# Autodesk Inventor assembly: sestava tělo estonsko s plechem
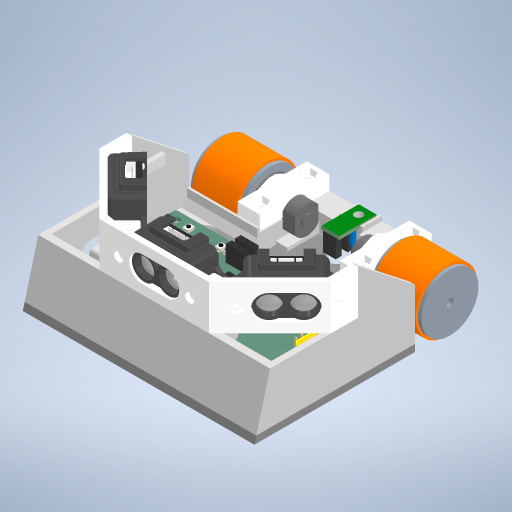
[picture p0: Inventor's stored thumbnail of the model, 512x512]
Saved by Autodesk Inventor 2024 (Build 280153000, 153)
## iProperties
Created: 2023-11-06
Part Number: sestava tělo estonsko s plechem
Document SubType Name: Assembly
Designer: jaryj
Author: jaryj
## Documents named in this file (9)
- C:\Users\Simak\OneDrive\Dokumenty\GitHub\RoboCop\- 3D -\wip\Tělo s plechem\sestava tělo estonsko s plechem.iam
- C:\Users\Simak\OneDrive\Dokumenty\GitHub\RoboCop\- 3D -\wip\Tělo s plechem\tělo estonsko s plechem.ipt
- C:\Users\Simak\OneDrive\Dokumenty\GitHub\RoboCop\- 3D -\el._parts\GA12-N20_Motor.ipt
- C:\Users\Simak\OneDrive\Dokumenty\GitHub\RoboCop\- 3D -\mech._parts\wheel+silicon.ipt
- C:\Users\Simak\OneDrive\Dokumenty\GitHub\RoboCop\- 3D -\wip\Sestava TF-Luna a držáku.iam
- C:\Users\Simak\OneDrive\Dokumenty\GitHub\RoboCop\- 3D -\mech._parts\plech.ipt
- C:\Users\Simak\OneDrive\Dokumenty\GitHub\RoboCop\- 3D -\el._parts\sumec_smd.iam
- C:\Users\Simak\OneDrive\Dokumenty\GitHub\RoboCop\- 3D -\mech._parts\motor_C_clamp_nutt.ipt
- C:\Users\Simak\OneDrive\Dokumenty\GitHub\RoboCop\- 3D -\el._parts\qre_module.ipt
## Components (11 placed, 8 different names)
1. tělo estonsko s plechem:1 — Vložit:2, Proti sobě:1, Vložit:3, Proti sobě:2, Proti sobě:5, Proti sobě:6, Proti sobě:10, Stejný směr:1, Proti sobě:11, Stejný směr:2, Proti sobě:12, Stejný směr:3, Proti sobě:13, Vložit:4, Vložit:5, Vložit:6, Vložit:7, Proti sobě:17, Vložit:8
2. GA12-N20_Motor:1 — Vložit:2, Proti sobě:1, Proti sobě:3, Proti sobě:14
3. GA12-N20_Motor:2 — Vložit:3, Proti sobě:2, Proti sobě:4, Proti sobě:15
4. wheel+silicon:1 — Proti sobě:4, Proti sobě:5
5. wheel+silicon:2 — Proti sobě:3, Proti sobě:6
6. Sestava TF-Luna a držáku:1 [sub-assembly] — Proti sobě:10, Stejný směr:1, Proti sobě:11
7. plech:1 — Stejný směr:2, Proti sobě:12, Stejný směr:3
8. sumec_smd:1 [sub-assembly] — Proti sobě:13, Vložit:4, Vložit:5
9. motor_C_clamp_nutt:1 — Proti sobě:15, Vložit:7
10. motor_C_clamp_nutt:2 — Proti sobě:14, Vložit:6
11. qre_module:1 — Proti sobě:17, Vložit:8
## Relationships (23: Mate 13, Insert 7, Flush 3)
- Vložit:2 [Insert]: tělo estonsko s plechem:1 ↔ GA12-N20_Motor:1
- Proti sobě:1 [Mate]: tělo estonsko s plechem:1 ↔ GA12-N20_Motor:1
- Vložit:3 [Insert]: tělo estonsko s plechem:1 ↔ GA12-N20_Motor:2
- Proti sobě:2 [Mate]: tělo estonsko s plechem:1 ↔ GA12-N20_Motor:2
- Proti sobě:3 [Mate]: GA12-N20_Motor:1 ↔ wheel+silicon:2
- Proti sobě:4 [Mate]: GA12-N20_Motor:2 ↔ wheel+silicon:1
- Proti sobě:5 [Mate] (0.5 mm): tělo estonsko s plechem:1 ↔ wheel+silicon:1
- Proti sobě:6 [Mate] (0.5 mm): tělo estonsko s plechem:1 ↔ wheel+silicon:2
- Proti sobě:10 [Mate]: tělo estonsko s plechem:1 ↔ Sestava TF-Luna a držáku:1
- Stejný směr:1 [Flush]: tělo estonsko s plechem:1 ↔ Sestava TF-Luna a držáku:1
- Proti sobě:11 [Mate] (-11.1058 mm): tělo estonsko s plechem:1 ↔ Sestava TF-Luna a držáku:1
- Stejný směr:2 [Flush]: tělo estonsko s plechem:1 ↔ plech:1
- Proti sobě:12 [Mate]: tělo estonsko s plechem:1 ↔ plech:1
- Stejný směr:3 [Flush]: tělo estonsko s plechem:1 ↔ plech:1
- Proti sobě:13 [Mate]: tělo estonsko s plechem:1 ↔ sumec_smd:1
- Vložit:4 [Insert]: tělo estonsko s plechem:1 ↔ sumec_smd:1
- Vložit:5 [Insert]: tělo estonsko s plechem:1 ↔ sumec_smd:1
- Proti sobě:14 [Mate]: GA12-N20_Motor:1 ↔ motor_C_clamp_nutt:2
- Vložit:6 [Insert]: tělo estonsko s plechem:1 ↔ motor_C_clamp_nutt:2
- Proti sobě:15 [Mate]: GA12-N20_Motor:2 ↔ motor_C_clamp_nutt:1
- Vložit:7 [Insert]: tělo estonsko s plechem:1 ↔ motor_C_clamp_nutt:1
- Proti sobě:17 [Mate]: tělo estonsko s plechem:1 ↔ qre_module:1
- Vložit:8 [Insert]: tělo estonsko s plechem:1 ↔ qre_module:1
